# Autodesk Inventor assembly: Montagem_v2
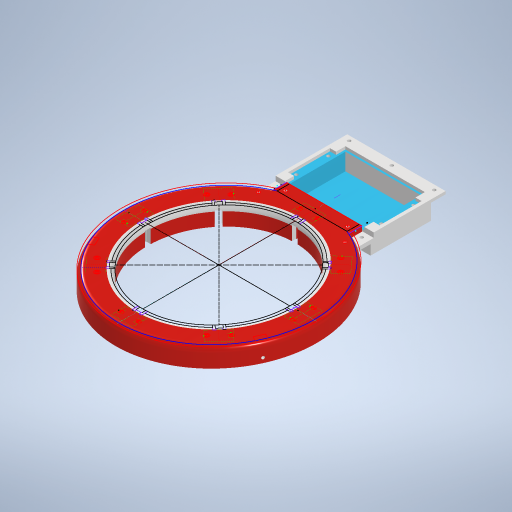
[picture p0: Inventor's stored thumbnail of the model, 512x512]
Saved by Autodesk Inventor 2024.3 (Build 283343000, 343)
## iProperties
Created: 2025-02-20
Part Number: Montagem_v2
Document SubType Name: Assembly
Designer: lostv
Author: lostv
## Documents named in this file (3)
- C:\Users\lostv\OneDrive\Área de Trabalho\Organizacao_Pesquisa\modelos_3D_IPT\Montagem_v2.iam
- C:\Users\lostv\OneDrive\Área de Trabalho\Organizacao_Pesquisa\modelos_3D_IPT\anel_v2.ipt
- C:\Users\lostv\OneDrive\Área de Trabalho\Organizacao_Pesquisa\modelos_3D_IPT\peca_principal_v2.ipt
## Components (2 placed, 2 different names)
1. anel_v2:1
2. peca_principal_v2:1
## Named parameters: Finish1_Area = 563.823, Finish2_Area = 68.7573, Finish3_Area = 283.285
note: some values were not read from the file. Shown as the stored number, unit unknown: "Finish1_Area", "Finish2_Area", "Finish3_Area".
